# Autodesk Inventor assembly: esc
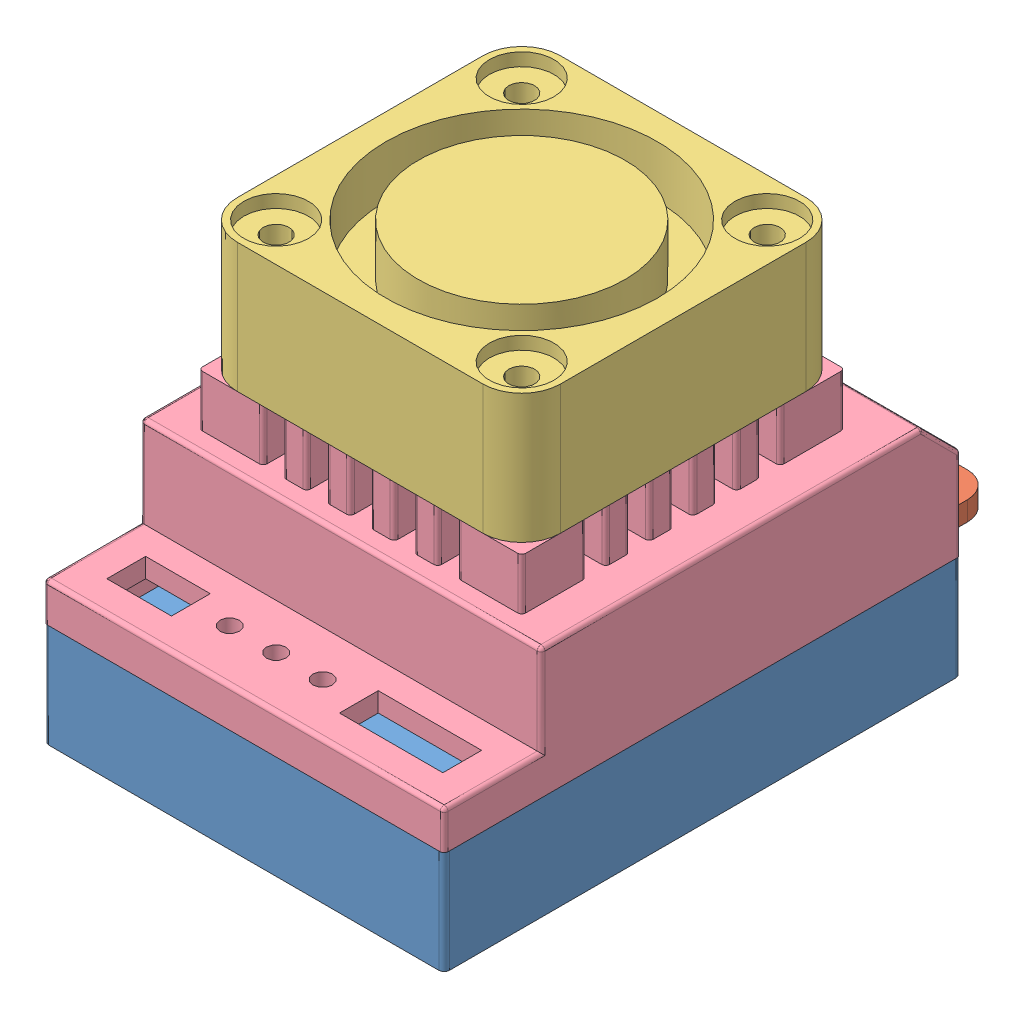
[picture p0: shaded view drawn from the shape stored in the file]
Saved by Autodesk Inventor 2021 (Build 250183000, 183)
## iProperties
Created: 2021-01-22
Part Number: esc
Document SubType Name: Assembly
Designer: User
Author: User
## Documents named in this file (5)
- D:\SynologyDrive\tcodev\tco-cad\common\esc\esc.iam
- D:\SynologyDrive\tcodev\tco-cad\common\esc\base.ipt
- D:\SynologyDrive\tcodev\tco-cad\common\esc\heatsink.ipt
- D:\SynologyDrive\tcodev\tco-cad\common\esc\board.ipt
- D:\SynologyDrive\tcodev\tco-cad\common\esc\fan.ipt
## Components (4 placed, 4 different names)
1. base:1 — Rigid:1, Mate:2
2. heatsink:1 — Rigid:1, Mate:1, Flush:1, Mate:3
3. board:1 — Mate:1, Mate:2, Flush:1
4. fan:1 — Mate:3
## Relationships (5: Mate 3, WeldJoint 1, Flush 1)
- Rigid:1 [WeldJoint]: base:1 ↔ heatsink:1
- Mate:1: heatsink:1 ↔ board:1
- Mate:2: base:1 ↔ board:1
- Flush:1 (-4.5 mm): heatsink:1 ↔ board:1
- Mate:3: heatsink:1 ↔ fan:1
